# Autodesk Inventor assembly: assem_finger_thumb_linact_v3
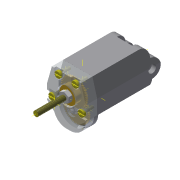
[picture p0: Inventor's stored thumbnail of the model, 180x180]
Saved by Autodesk Inventor 2014 (Build 180170000, 170)
## iProperties
Created: 2015-05-30
Part Number: assem_finger_thumb_linact_v3
Document SubType Name: Assembly
Designer: Martin
Author: Martin
## Documents named in this file (11)
- C:\Users\Martin\Dropbox\biohand-mec\biohand_v1\fingers\thumb\assem_finger_thumb_linact_v3.iam
- C:\Users\Martin\Dropbox\biohand-mec\biohand_v1\fingers\thumb\linact_thumb_cage_v2.ipt
- C:\Users\Martin\Dropbox\biohand-mec\biohand_v1\misc\motor_servo.ipt
- C:\Users\Martin\Dropbox\biohand-mec\biohand_v1\fingers\thumb\linact_thumb_front_v2.ipt
- C:\Users\Martin\Dropbox\biohand-mec\biohand_v1\misc\servo_gear_1.ipt
- C:\Users\Martin\Dropbox\biohand-mec\biohand_v1\misc\servo_gear_2.ipt
- C:\Users\Martin\Dropbox\biohand-mec\biohand_v1\misc\m2_8_screw.ipt
- C:\Users\Martin\Dropbox\biohand-mec\biohand_v1\misc\m3_30_screw.ipt
- C:\Users\Martin\Dropbox\biohand-mec\biohand_v1\misc\m3_nut.ipt
- C:\Users\Martin\Dropbox\biohand-mec\biohand_v1\misc\m3_20_screw.ipt
- C:\Users\Martin\Dropbox\biohand-mec\biohand_v1\misc\servo_small_dowel.ipt
## Components (13 placed, 10 different names)
1. linact_thumb_cage_v2:1 — Insert:1, Mate:1, Flush:1, Insert:2
2. motor_servo:1 — Insert:1, Mate:1
3. linact_thumb_front_v2:1 — Flush:2, Insert:3, Insert:4, Insert:5, Insert:6, Insert:7, Insert:11
4. servo_gear_1:1 — Insert:2
5. servo_gear_2:1 — Insert:3, Insert:8, Insert:9, Insert:10
6. m2_8_screw:1 — Insert:6
7. m2_8_screw:2 — Insert:7
8. m2_8_screw:3 — Insert:4
9. m2_8_screw:4 — Insert:5
10. m3_30_screw:1 — Insert:8
11. m3_nut:1 — Insert:9
12. m3_20_screw:1 — Insert:10
13. servo_small_dowel:1 — Insert:11
## Relationships (14: Insert 11, Flush 2, Mate 1)
- Insert:1: linact_thumb_cage_v2:1 ↔ motor_servo:1
- Mate:1: linact_thumb_cage_v2:1 ↔ motor_servo:1
- Flush:1 (2.8 mm): linact_thumb_cage_v2:1
- Flush:2: linact_thumb_front_v2:1
- Insert:2 (0.25 mm): linact_thumb_cage_v2:1 ↔ servo_gear_1:1
- Insert:3 (0.25 mm): linact_thumb_front_v2:1 ↔ servo_gear_2:1
- Insert:4: linact_thumb_front_v2:1 ↔ m2_8_screw:3
- Insert:5: linact_thumb_front_v2:1 ↔ m2_8_screw:4
- Insert:6: linact_thumb_front_v2:1 ↔ m2_8_screw:1
- Insert:7: linact_thumb_front_v2:1 ↔ m2_8_screw:2
- Insert:8: servo_gear_2:1 ↔ m3_30_screw:1
- Insert:9: servo_gear_2:1 ↔ m3_nut:1
- Insert:10: servo_gear_2:1 ↔ m3_20_screw:1
- Insert:11 (-0.45 mm): linact_thumb_front_v2:1 ↔ servo_small_dowel:1
